# Autodesk Inventor assembly: test
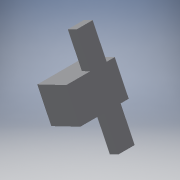
[picture p0: Inventor's stored thumbnail of the model, 180x180]
Saved by Autodesk Inventor 2019 (Build 230136000, 136)
## iProperties
Created: 2024-11-10
Part Number: test
Material: Generisch
Document SubType Name: Assembly
Designer: nic
Author: nic
## Documents named in this file (3)
- C:\Users\Nicolas Frick\Sync\OneDrive\wtm\nicol_rh8d\inventor\test.iam
- C:\Users\Nicolas Frick\Sync\OneDrive\wtm\nias\nias_description\inventor_files\w.ipt
- C:\Users\Nicolas Frick\Sync\OneDrive\wtm\nias\nias_description\inventor_files\f2.ipt
## Components (2 placed, 2 different names)
1. w:1 — Passend:1, Fluchtend:1, Passend:2, Fluchtend:2, Winkel:1
2. f2:1 — Passend:2, Fluchtend:2, Winkel:1
## Relationships (5: Mate 2, Flush 2, Angle 1)
- Passend:1 [Mate]: w:1
- Fluchtend:1 [Flush]: w:1
- Passend:2 [Mate]: w:1 ↔ f2:1
- Fluchtend:2 [Flush]: w:1 ↔ f2:1
- Winkel:1 [Angle] (0 deg): w:1 ↔ f2:1
